# Autodesk Inventor assembly: UpperBackLink
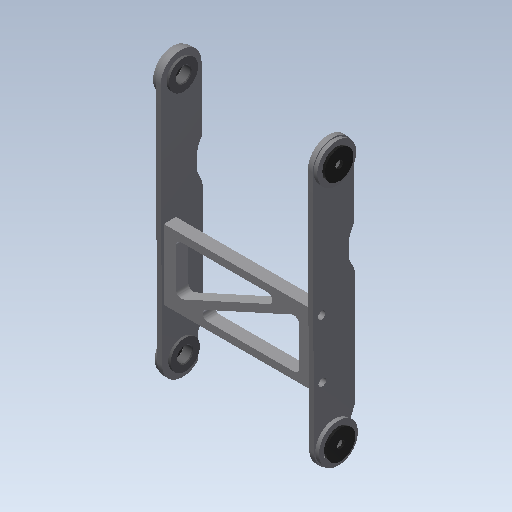
[picture p0: Inventor's stored thumbnail of the model, 512x512]
Saved by Autodesk Inventor 2020.4 (Build 244396000, 396)
## iProperties
Created: 2016-08-23
Part Number: UpperBackLink
Material: 一般
Document SubType Name: Assembly
Designer: hiro
Mass: 25.265 g
Surface Area: 146.992 cm^2
Volume: 11.3922 cm^3
Density: 2.21774 g/cm^3
Author: hiro
## Documents named in this file (6)
- C:\Users\Masato\Documents\Inventor\CIT Brains_Inventor\OpenPlatform_ver3_0\下半身\リンク\UpperBackLink.iam
- C:\Users\Masato\Documents\Inventor\CIT Brains_Inventor\OpenPlatform_ver3_0\下半身\リンク\リンク_メインフレーム_6_1.ipt
- C:\Users\Masato\Documents\Inventor\CIT Brains_Inventor\OpenPlatform_ver3_0\下半身\リンク\リンク_ふくらはぎ_サブフレーム_1_2.ipt
- C:\Users\Masato\Documents\Inventor\CIT Brains_Inventor\OpenPlatform_ver3_0\Ready_Made\UUW-0312-10BH.ipt
- C:\Users\Masato\Documents\Inventor\CIT Brains_Inventor\OpenPlatform_ver3_0\Ready_Made\80F-0603.ipt
- C:\Users\Masato\Documents\Inventor\CIT Brains_Inventor\OpenPlatform_ver3_0\Ready_Made\LFW-0815.ipt
## Components (15 placed, 5 different names)
1. リンク_メインフレーム_6_1:1 — 挿入:21, 挿入:22, 挿入:27, 挿入:28, 挿入:33, 挿入:34
2. リンク_メインフレーム_6_1:2 — 挿入:23, 挿入:24, 挿入:25, 挿入:26, 挿入:35, 挿入:36
3. UUW-0312-10BH:1 — 挿入:29
4. UUW-0312-10BH:2 — 挿入:30
5. UUW-0312-10BH:3 — 挿入:31
6. UUW-0312-10BH:4 — 挿入:32
7. リンク_ふくらはぎ_サブフレーム_1_2:1 — 挿入:21, 挿入:22, 挿入:23, 挿入:24
8. 80F-0603:1 — 挿入:25
9. 80F-0603:2 — 挿入:26
10. 80F-0603:3 — 挿入:27
11. 80F-0603:4 — 挿入:28
12. LFW-0815:1 — 挿入:32, 挿入:35
13. LFW-0815:2 — 挿入:31, 挿入:36
14. LFW-0815:3 — 挿入:30, 挿入:33
15. LFW-0815:4 — 挿入:29, 挿入:34
## Relationships (16: Insert 16)
- 挿入:21 [Insert]: リンク_メインフレーム_6_1:1 ↔ リンク_ふくらはぎ_サブフレーム_1_2:1
- 挿入:22 [Insert]: リンク_メインフレーム_6_1:1 ↔ リンク_ふくらはぎ_サブフレーム_1_2:1
- 挿入:23 [Insert]: リンク_メインフレーム_6_1:2 ↔ リンク_ふくらはぎ_サブフレーム_1_2:1
- 挿入:24 [Insert]: リンク_メインフレーム_6_1:2 ↔ リンク_ふくらはぎ_サブフレーム_1_2:1
- 挿入:25 [Insert]: リンク_メインフレーム_6_1:2 ↔ 80F-0603:1
- 挿入:26 [Insert]: リンク_メインフレーム_6_1:2 ↔ 80F-0603:2
- 挿入:27 [Insert]: リンク_メインフレーム_6_1:1 ↔ 80F-0603:3
- 挿入:28 [Insert]: リンク_メインフレーム_6_1:1 ↔ 80F-0603:4
- 挿入:29 [Insert]: UUW-0312-10BH:1 ↔ LFW-0815:4
- 挿入:30 [Insert]: UUW-0312-10BH:2 ↔ LFW-0815:3
- 挿入:31 [Insert]: UUW-0312-10BH:3 ↔ LFW-0815:2
- 挿入:32 [Insert]: UUW-0312-10BH:4 ↔ LFW-0815:1
- 挿入:33 [Insert]: リンク_メインフレーム_6_1:1 ↔ LFW-0815:3
- 挿入:34 [Insert]: リンク_メインフレーム_6_1:1 ↔ LFW-0815:4
- 挿入:35 [Insert]: リンク_メインフレーム_6_1:2 ↔ LFW-0815:1
- 挿入:36 [Insert]: リンク_メインフレーム_6_1:2 ↔ LFW-0815:2
